# Autodesk Inventor assembly: Res
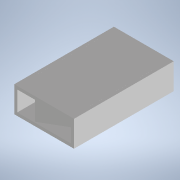
[picture p0: Inventor's stored thumbnail of the model, 180x180]
Saved by Autodesk Inventor 2020 (Build 240168000, 168)
## iProperties
Created: 2021-02-07
Part Number: Res
Document SubType Name: Assembly
Designer: moham
Author: moham
## Documents named in this file (4)
- D:\Projects\MCT 131\The project\Resevoir\Res.iam
- D:\Projects\MCT 131\The project\Resevoir\Frontandback_2.ipt
- D:\Projects\MCT 131\The project\Resevoir\Sides_2.ipt
- D:\Projects\MCT 131\The project\Resevoir\zigzags.ipt
## Components (5 placed, 3 different names)
1. Frontandback_2:1 — Mate:1, Flush:1, Flush:2, Mate:3, Mate:4
2. Sides_2:1 — Mate:1, Flush:1, Flush:2, Angle:1, Mate:5, Flush:3, Flush:4
3. Frontandback_2:2 — Mate:5, Flush:3, Flush:4, Mate:6, Flush:5, Flush:6
4. Sides_2:2 — Mate:6, Flush:5, Flush:6
5. zigzags:1 — Mate:3, Angle:1, Mate:4
## Relationships (12: Flush 6, Mate 5, Angle 1)
- Mate:1: Frontandback_2:1 ↔ Sides_2:1
- Flush:1: Frontandback_2:1 ↔ Sides_2:1
- Flush:2: Frontandback_2:1 ↔ Sides_2:1
- Mate:3: Frontandback_2:1 ↔ zigzags:1
- Angle:1 (60 deg): Sides_2:1 ↔ zigzags:1
- Mate:4: Frontandback_2:1 ↔ zigzags:1
- Mate:5: Sides_2:1 ↔ Frontandback_2:2
- Flush:3: Sides_2:1 ↔ Frontandback_2:2
- Flush:4: Sides_2:1 ↔ Frontandback_2:2
- Mate:6: Frontandback_2:2 ↔ Sides_2:2
- Flush:5: Frontandback_2:2 ↔ Sides_2:2
- Flush:6: Frontandback_2:2 ↔ Sides_2:2
